# Autodesk Inventor assembly: Turret Assembly
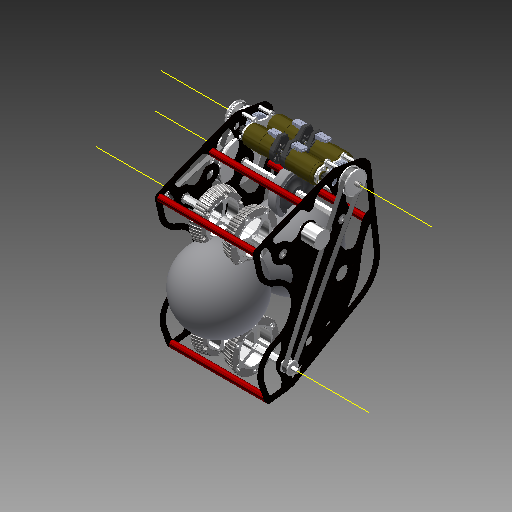
[picture p0: Inventor's stored thumbnail of the model, 512x512]
Saved by Autodesk Inventor 2019.4 (Build 234330000, 330)
## iProperties
Created: 2020-01-16
Part Number: Turret Assembly
Document SubType Name: Assembly
Designer: admin
Mass: 8414.5 g
Surface Area: 10801.7 cm^2
Volume: 8393.65 cm^3
Density: 1.00248 g/cm^3
Author: admin
## Documents named in this file (21)
- C:\Users\Mark\Desktop\7738 Helion Engineering\7738-2020\Robot V2\Turret\Turret Assembly.iam
- C:\Users\Mark\Desktop\7738 Helion Engineering\7738-2020\Robot V2\Turret\Flywheel Half.ipt
- C:\Users\Mark\Desktop\7738 Helion Engineering\7738-2020\Robot V2\Turret\Colson_Performa_4_x_0_875_1_2_Hex_bore_217-4049.ipt
- C:\Users\Mark\Desktop\7738 Helion Engineering\7738-2020\Robot V2\Turret\Shooter Side Plate.ipt
- C:\Users\Mark\Desktop\7738 Helion Engineering\7738-2020\Power Cell.ipt
- C:\Users\Mark\Desktop\7738 Helion Engineering\7738-2020\Robot V2\Turret\775\775pro_775pro_Connect_and_8T_Pinion_217-6459.iam
- C:\Users\Mark\Desktop\7738 Helion Engineering\7738-2020\Robot V2\Turret\36t_Aluminum_Spur_Gear_20_DP_1_2_Hex_Bore_217-3214.ipt
- C:\Users\Mark\Desktop\7738 Helion Engineering\7738-2020\Robot V2\Turret\F6800.ipt
- C:\Users\Mark\Desktop\7738 Helion Engineering\7738-2020\Robot V2\Turret\Turret Assembly\Design Accelerator\Synchronous Belts Transmission10.iam
- C:\Users\Mark\Desktop\7738 Helion Engineering\7738-2020\Robot V2\Turret\Motor Bracket.ipt
- C:\Users\Mark\Desktop\7738 Helion Engineering\7738-2020\Robot V2\Turret\F6700ZZ Bearing.ipt
- C:\Users\Mark\Desktop\7738 Helion Engineering\7738-2020\Robot V2\Turret\Motor Bracket Spacer.ipt
- C:\Users\Mark\Desktop\7738 Helion Engineering\7738-2020\Robot V2\Turret\Gearbox Axle.ipt
- C:\Users\Mark\Desktop\7738 Helion Engineering\7738-2020\Robot V2\Turret\Flywheel Axle.ipt
- C:\Users\Mark\Desktop\7738 Helion Engineering\7738-2020\Robot V2\Turret\Shooter Spacer.ipt
- C:\Users\Mark\Desktop\7738 Helion Engineering\7738-2020\Robot V2\Turret\EB38S6 Encoder.ipt
- C:\Users\Mark\Desktop\7738 Helion Engineering\7738-2020\Robot V2\Turret\Turret Assembly\Design Accelerator\Key Connection1.iam
- C:\Users\Mark\Desktop\7738 Helion Engineering\7738-2020\Robot V2\Turret\Turret Assembly\Design Accelerator\Synchronous Belts Transmission11.iam
- C:\Users\Mark\Desktop\7738 Helion Engineering\7738-2020\Robot V2\Turret\Turret Assembly\Design Accelerator\Synchronous Belts Transmission12.iam
- C:\Users\Mark\Desktop\7738 Helion Engineering\7738-2020\Robot V2\Turret\Turret Assembly\Design Accelerator\Key Connection5.iam
- C:\Users\Mark\Desktop\7738 Helion Engineering\7738-2020\Robot V2\Turret\Flywheel Mass.ipt
## Components (55 placed, 17 different names)
1. Shooter Side Plate:1 — Mate:34, Mate:38, Mate:39, Mate:43, Mate:45, Mate:49, Mate:68, Mate:69, Mate:70, Mate:71, Mate:72, Mate:78, Mate:79, Mate:84, Mate:85, Mate:88, Mate:89, Mate:149, Mate:150, Mate:151, Mate:152, Mate:168, Mate:170, Mate:173, Mate:175, Mate:176, Mate:177, Mate:178, Mate:179
2. Colson_Performa_4_x_0_875_1_2_Hex_bore_217-4049:3 — Mate:45, Mate:46
3. Flywheel Half:11 — Mate:35, Mate:36, Mate:37, Mate:38, Mate:47, Mate:186, Mate:189, Flush:12
4. Flywheel Half:12 — Mate:35, Mate:36, Mate:184, Mate:185, Flush:9
5. Flywheel Half:13 — Mate:42, Mate:43, Mate:48, Mate:187, Mate:190, Flush:11
6. Flywheel Half:14 — Mate:188, Mate:191, Flush:10
7. Power Cell:1 — Mate:44
8. Shooter Side Plate:2 — Mate:47, Mate:48, Mate:49, Mate:73, Mate:74, Mate:75, Mate:76, Mate:77, Mate:80, Mate:81, Mate:82, Mate:83, Mate:86, Mate:87, Mate:139, Mate:140, Mate:141, Mate:142, Mate:166, Mate:171, Mate:172, Mate:174
9. 775pro_775pro_Connect_and_8T_Pinion_217-6459:5 [sub-assembly] — Flush:3, Mate:69, Mate:95, Mate:96, Mate:193
10. 36t_Aluminum_Spur_Gear_20_DP_1_2_Hex_Bore_217-3214:3 — Mate:68, Flush:3, Flush:4
11. F6800:7 — Mate:71, Mate:72
12. 775pro_775pro_Connect_and_8T_Pinion_217-6459:6 [sub-assembly] — Flush:4, Mate:70, Mate:144, Mate:192
13. 775pro_775pro_Connect_and_8T_Pinion_217-6459:7 [sub-assembly] — Flush:5, Mate:75, Mate:134, Mate:195
14. 36t_Aluminum_Spur_Gear_20_DP_1_2_Hex_Bore_217-3214:4 — Mate:73, Flush:5, Flush:6
15. 775pro_775pro_Connect_and_8T_Pinion_217-6459:8 [sub-assembly] — Flush:6, Mate:74, Mate:92, Mate:93, Mate:194
16. F6800:8 — Mate:76, Mate:77
17. F6800:9 — Mate:78, Mate:79, Mate:181, Mate:182
18. F6800:10 — Mate:80, Mate:81
19. Synchronous Belts Transmission:4 [sub-assembly]
20. F6800:11 — Mate:82, Mate:83, Mate:128, Mate:129, Mate:167
21. F6800:12 — Mate:84, Mate:85
22. F6800:13 — Mate:86, Mate:87
23. F6800:14 — Mate:88, Mate:89, Mate:130, Mate:131, Mate:169
24. Power Cell:2 — Mate:90, Mate:91
25. Motor Bracket:1 — Mate:92, Mate:93, Mate:118, Mate:119, Mate:134, Mate:135, Mate:136, Mate:137, Mate:138, Mate:143, Mate:194, Mate:195
26. Motor Bracket:2 — Mate:95, Mate:96, Mate:120, Mate:121, Mate:144, Mate:145, Mate:146, Mate:147, Mate:148, Mate:153, Mate:192, Mate:193
27. Motor Bracket Spacer:1 — Mate:136, Mate:139, Mate:143
28. Motor Bracket Spacer:2 — Mate:137, Mate:141
29. Motor Bracket Spacer:3 — Mate:138, Mate:142
30. Motor Bracket Spacer:4 — Mate:135, Mate:140
31. Motor Bracket Spacer:5 — Mate:146, Mate:149
32. Motor Bracket Spacer:6 — Mate:147, Mate:151
33. Motor Bracket Spacer:7 — Mate:148, Mate:152
34. Motor Bracket Spacer:8 — Mate:145, Mate:150, Mate:153
35. F6700ZZ Bearing:3 — Mate:118, Mate:119, Mate:122, Mate:123
36. F6700ZZ Bearing:4 — Mate:120, Mate:121, Mate:126, Mate:127
37. Gearbox Axle:1 — Mate:122, Mate:123
38. Gearbox Axle:2 — Mate:126, Mate:127, Flush:13, Angle:5, Mate:196
39. Flywheel Axle:1 — Mate:128, Mate:129
40. Flywheel Axle:2 — Mate:130, Mate:131
41. EB38S6 Encoder:1 — Mate:166, Mate:167, Mate:171
42. EB38S6 Encoder:2 — Mate:168, Mate:169, Mate:170
43. Shooter Spacer:3 — Mate:176, Mate:177
44. Shooter Spacer:4 — Mate:174, Mate:175
45. Shooter Spacer:5 — Mate:172, Mate:173
46. Shooter Spacer:6 — Mate:178, Mate:179
47. Key Connection:1 [sub-assembly] — Flush:13, Angle:5, Mate:196
48. Flywheel Axle:3 — Mate:181, Mate:182, Flush:14, Angle:6, Mate:197
49. Synchronous Belts Transmission:5 [sub-assembly]
50. Synchronous Belts Transmission:6 [sub-assembly]
51. Key Connection:2 [sub-assembly] — Flush:14, Angle:6, Mate:197
52. Flywheel Mass:1 — Mate:184, Mate:185, Flush:9
53. Flywheel Mass:2 — Mate:186, Mate:189, Flush:12
54. Flywheel Mass:3 — Mate:187, Mate:190, Flush:11
55. Flywheel Mass:4 — Mate:188, Mate:191, Flush:10
## Relationships (118: Mate 106, Flush 10, Angle 2)
- Mate:34 (114.3 mm): Shooter Side Plate:1
- Mate:35: Flywheel Half:11 ↔ Flywheel Half:12
- Mate:36 (50 mm): Flywheel Half:11 ↔ Flywheel Half:12
- Mate:37 (25 mm): Flywheel Half:11
- Mate:38: Shooter Side Plate:1 ↔ Flywheel Half:11
- Mate:39: Shooter Side Plate:1
- [Mate]: Flywheel Half:13 ↔ Flywheel Half:14
- [Mate] (50 mm): Flywheel Half:13 ↔ Flywheel Half:14
- Mate:42 (25 mm): Flywheel Half:13
- Mate:43: Shooter Side Plate:1 ↔ Flywheel Half:13
- Mate:44: Power Cell:1
- Mate:45: Shooter Side Plate:1 ↔ Colson_Performa_4_x_0_875_1_2_Hex_bore_217-4049:3
- Mate:46: Colson_Performa_4_x_0_875_1_2_Hex_bore_217-4049:3
- Mate:47: Flywheel Half:11 ↔ Shooter Side Plate:2
- Mate:48: Flywheel Half:13 ↔ Shooter Side Plate:2
- Mate:49 (228.6 mm): Shooter Side Plate:1 ↔ Shooter Side Plate:2
- Mate:68: Shooter Side Plate:1 ↔ 36t_Aluminum_Spur_Gear_20_DP_1_2_Hex_Bore_217-3214:3
- Flush:3 (-4 mm): 775pro_775pro_Connect_and_8T_Pinion_217-6459:5 ↔ 36t_Aluminum_Spur_Gear_20_DP_1_2_Hex_Bore_217-3214:3
- Mate:69: Shooter Side Plate:1 ↔ 775pro_775pro_Connect_and_8T_Pinion_217-6459:5
- Flush:4 (-4 mm): 36t_Aluminum_Spur_Gear_20_DP_1_2_Hex_Bore_217-3214:3 ↔ 775pro_775pro_Connect_and_8T_Pinion_217-6459:6
- Mate:70: Shooter Side Plate:1 ↔ 775pro_775pro_Connect_and_8T_Pinion_217-6459:6
- Mate:71 (0.2 mm): Shooter Side Plate:1 ↔ F6800:7
- Mate:72: Shooter Side Plate:1 ↔ F6800:7
- Mate:73: Shooter Side Plate:2 ↔ 36t_Aluminum_Spur_Gear_20_DP_1_2_Hex_Bore_217-3214:4
- Flush:5 (-4 mm): 775pro_775pro_Connect_and_8T_Pinion_217-6459:7 ↔ 36t_Aluminum_Spur_Gear_20_DP_1_2_Hex_Bore_217-3214:4
- Flush:6 (-4 mm): 36t_Aluminum_Spur_Gear_20_DP_1_2_Hex_Bore_217-3214:4 ↔ 775pro_775pro_Connect_and_8T_Pinion_217-6459:8
- Mate:74: Shooter Side Plate:2 ↔ 775pro_775pro_Connect_and_8T_Pinion_217-6459:8
- Mate:75: Shooter Side Plate:2 ↔ 775pro_775pro_Connect_and_8T_Pinion_217-6459:7
- Mate:76 (0.2 mm): Shooter Side Plate:2 ↔ F6800:8
- Mate:77: Shooter Side Plate:2 ↔ F6800:8
- Mate:78 (0.2 mm): Shooter Side Plate:1 ↔ F6800:9
- Mate:79: Shooter Side Plate:1 ↔ F6800:9
- Mate:80 (0.2 mm): Shooter Side Plate:2 ↔ F6800:10
- Mate:81: Shooter Side Plate:2 ↔ F6800:10
- Mate:82 (0.2 mm): Shooter Side Plate:2 ↔ F6800:11
- Mate:83: Shooter Side Plate:2 ↔ F6800:11
- Mate:84 (0.2 mm): Shooter Side Plate:1 ↔ F6800:12
- Mate:85: Shooter Side Plate:1 ↔ F6800:12
- Mate:86 (0.2 mm): Shooter Side Plate:2 ↔ F6800:13
- Mate:87: Shooter Side Plate:2 ↔ F6800:13
- Mate:88 (0.2 mm): Shooter Side Plate:1 ↔ F6800:14
- Mate:89: Shooter Side Plate:1 ↔ F6800:14
- Mate:90: Power Cell:2
- Mate:91: Power Cell:2
- Mate:92: 775pro_775pro_Connect_and_8T_Pinion_217-6459:8 ↔ Motor Bracket:1
- Mate:93: 775pro_775pro_Connect_and_8T_Pinion_217-6459:8 ↔ Motor Bracket:1
- Mate:95: 775pro_775pro_Connect_and_8T_Pinion_217-6459:5 ↔ Motor Bracket:2
- Mate:96: 775pro_775pro_Connect_and_8T_Pinion_217-6459:5 ↔ Motor Bracket:2
- Mate:118: Motor Bracket:1 ↔ F6700ZZ Bearing:3
- Mate:119 (0.2 mm): Motor Bracket:1 ↔ F6700ZZ Bearing:3
- Mate:120: Motor Bracket:2 ↔ F6700ZZ Bearing:4
- Mate:121 (0.2 mm): Motor Bracket:2 ↔ F6700ZZ Bearing:4
- Mate:122: F6700ZZ Bearing:3 ↔ Gearbox Axle:1
- Mate:123 (0.1 mm): F6700ZZ Bearing:3 ↔ Gearbox Axle:1
- Mate:126: F6700ZZ Bearing:4 ↔ Gearbox Axle:2
- Mate:127 (0.1 mm): F6700ZZ Bearing:4 ↔ Gearbox Axle:2
- Mate:128: F6800:11 ↔ Flywheel Axle:1
- Mate:129: F6800:11 ↔ Flywheel Axle:1
- Mate:130: F6800:14 ↔ Flywheel Axle:2
- Mate:131: F6800:14 ↔ Flywheel Axle:2
- Mate:134: 775pro_775pro_Connect_and_8T_Pinion_217-6459:7 ↔ Motor Bracket:1
- Mate:135: Motor Bracket:1 ↔ Motor Bracket Spacer:4
- Mate:136: Motor Bracket:1 ↔ Motor Bracket Spacer:1
- Mate:137: Motor Bracket:1 ↔ Motor Bracket Spacer:2
- Mate:138: Motor Bracket:1 ↔ Motor Bracket Spacer:3
- Mate:139: Shooter Side Plate:2 ↔ Motor Bracket Spacer:1
- Mate:140: Shooter Side Plate:2 ↔ Motor Bracket Spacer:4
- Mate:141: Shooter Side Plate:2 ↔ Motor Bracket Spacer:2
- Mate:142: Shooter Side Plate:2 ↔ Motor Bracket Spacer:3
- Mate:143: Motor Bracket:1 ↔ Motor Bracket Spacer:1
- Mate:144: 775pro_775pro_Connect_and_8T_Pinion_217-6459:6 ↔ Motor Bracket:2
- Mate:145: Motor Bracket:2 ↔ Motor Bracket Spacer:8
- Mate:146: Motor Bracket:2 ↔ Motor Bracket Spacer:5
- Mate:147: Motor Bracket:2 ↔ Motor Bracket Spacer:6
- Mate:148: Motor Bracket:2 ↔ Motor Bracket Spacer:7
- Mate:149: Shooter Side Plate:1 ↔ Motor Bracket Spacer:5
- Mate:150: Shooter Side Plate:1 ↔ Motor Bracket Spacer:8
- Mate:151: Shooter Side Plate:1 ↔ Motor Bracket Spacer:6
- Mate:152: Shooter Side Plate:1 ↔ Motor Bracket Spacer:7
- Mate:153: Motor Bracket:2 ↔ Motor Bracket Spacer:8
- Mate:166: Shooter Side Plate:2 ↔ EB38S6 Encoder:1
- Mate:167 (63.4 mm): F6800:11 ↔ EB38S6 Encoder:1
- Mate:168: Shooter Side Plate:1 ↔ EB38S6 Encoder:2
- Mate:169 (63.4 mm): F6800:14 ↔ EB38S6 Encoder:2
- Mate:170: Shooter Side Plate:1 ↔ EB38S6 Encoder:2
- Mate:171: Shooter Side Plate:2 ↔ EB38S6 Encoder:1
- Mate:172: Shooter Side Plate:2 ↔ Shooter Spacer:5
- Mate:173: Shooter Side Plate:1 ↔ Shooter Spacer:5
- Mate:174: Shooter Side Plate:2 ↔ Shooter Spacer:4
- Mate:175: Shooter Side Plate:1 ↔ Shooter Spacer:4
- Mate:176: Shooter Side Plate:1 ↔ Shooter Spacer:3
- Mate:177: Shooter Side Plate:1 ↔ Shooter Spacer:3
- Mate:178: Shooter Side Plate:1 ↔ Shooter Spacer:6
- Mate:179: Shooter Side Plate:1 ↔ Shooter Spacer:6
- Mate:181: F6800:9 ↔ Flywheel Axle:3
- Mate:182: F6800:9 ↔ Flywheel Axle:3
- Mate:184: Flywheel Half:12 ↔ Flywheel Mass:1
- Mate:185: Flywheel Half:12 ↔ Flywheel Mass:1
- Flush:9: Flywheel Half:12 ↔ Flywheel Mass:1
- Mate:186: Flywheel Half:11 ↔ Flywheel Mass:2
- Mate:187: Flywheel Half:13 ↔ Flywheel Mass:3
- Mate:188: Flywheel Half:14 ↔ Flywheel Mass:4
- Mate:189: Flywheel Half:11 ↔ Flywheel Mass:2
- Mate:190: Flywheel Half:13 ↔ Flywheel Mass:3
- Mate:191: Flywheel Half:14 ↔ Flywheel Mass:4
- Flush:10: Flywheel Half:14 ↔ Flywheel Mass:4
- Flush:11: Flywheel Half:13 ↔ Flywheel Mass:3
- Flush:12: Flywheel Half:11 ↔ Flywheel Mass:2
- Mate:192: 775pro_775pro_Connect_and_8T_Pinion_217-6459:6 ↔ Motor Bracket:2
- Mate:193: 775pro_775pro_Connect_and_8T_Pinion_217-6459:5 ↔ Motor Bracket:2
- Mate:194: 775pro_775pro_Connect_and_8T_Pinion_217-6459:8 ↔ Motor Bracket:1
- Mate:195: 775pro_775pro_Connect_and_8T_Pinion_217-6459:7 ↔ Motor Bracket:1
- Flush:13 (11.1961 mm): Gearbox Axle:2 ↔ Key Connection:1
- Angle:5 (0 deg): Gearbox Axle:2 ↔ Key Connection:1
- Mate:196: Gearbox Axle:2 ↔ Key Connection:1
- Flush:14 (1.1329 mm): Flywheel Axle:3 ↔ Key Connection:2
- Angle:6 (0 deg): Flywheel Axle:3 ↔ Key Connection:2
- Mate:197: Flywheel Axle:3 ↔ Key Connection:2
## Named parameters: d73_d68 = 0 mm, d74_d69 = 50 mm
